# Autodesk Inventor assembly: Board
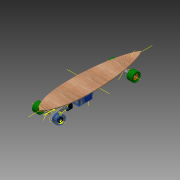
[picture p0: Inventor's stored thumbnail of the model, 180x180]
Saved by Autodesk Inventor 2015 (Build 190159000, 159)
## iProperties
Created: 2014-05-13
Part Number: Board
Document SubType Name: Assembly
Designer: dliu
Author: dliu
## Documents named in this file (9)
- C:\Users\dliu\Dropbox\dbhome\electric-longboard\dliu\DLiu Board.iam
- C:\Users\dliu\Dropbox\dbhome\electric-longboard\dliu\Board\Deck Pintail 9x37.iam
- C:\Users\dliu\Dropbox\dbhome\electric-longboard\dliu\Mount\Truck Caliber50 9in.iam
- C:\Users\dliu\Dropbox\dbhome\electric-longboard\dliu\Board\Wheel Blank Pro 83mm.ipt
- C:\Users\dliu\Dropbox\dbhome\electric-longboard\dliu\Mount\Mount.iam
- C:\Users\dliu\Dropbox\dbhome\electric-longboard\dliu\Electronics\Motor SK3 5065 275KV.ipt
- C:\Users\dliu\Dropbox\dbhome\electric-longboard\dliu\Pulleys\a_6a25m012df1506.ipt
- C:\Users\dliu\Dropbox\dbhome\electric-longboard\dliu\Wheel Insert\Wheel Insert Test Fit.iam
- C:\Users\dliu\Dropbox\dbhome\electric-longboard\dliu\Electronics\ElectronicsBox with components.iam
## Components (12 placed, 8 different names)
1. Deck Pintail 9x37:1 [sub-assembly] — Mate:1, Flush:3, Insert:3, Insert:4, Mate:19, Mate:20, Mate:21, Mate:26, Mate:28, Mate:29, Mate:30, Mate:31
2. Truck Caliber50 9in:1 [sub-assembly] — Mate:2, Mate:3, Mate:8, Mate:9, Mate:26, Mate:28, Mate:29, Mate:30, Mate:31
3. Truck Caliber50 9in:2 [sub-assembly] — Insert:3, Insert:4, Mate:4, Mate:5, Mate:6, Mate:7, Mate:12, Mate:13, Mate:14, Mate:19, Mate:20, Mate:21, Mate:34, Mate:35
4. Wheel Blank Pro 83mm:1 — Mate:2, Mate:3
5. Wheel Blank Pro 83mm:2 — Mate:8, Mate:9
6. Wheel Blank Pro 83mm:3 — Mate:6, Mate:7
7. Wheel Blank Pro 83mm:4 — Mate:4, Mate:5
8. Mount:1 [sub-assembly] — Mate:12, Mate:13, Mate:14, Mate:17, Mate:18, Mate:24
9. Motor SK3 5065 275KV:1 — Mate:17, Mate:18, Mate:22
10. a_6a25m012df1506:1 — Mate:22, Mate:24
11. Wheel Insert Test Fit:1 [sub-assembly] — Mate:34, Mate:35
12. ElectronicsBox with components:1 [sub-assembly]
## Relationships (29: Mate 26, Insert 2, Flush 1)
- Mate:1: Deck Pintail 9x37:1
- Flush:3: Deck Pintail 9x37:1
- Insert:3 (6.35 mm): Deck Pintail 9x37:1 ↔ Truck Caliber50 9in:2
- Insert:4 (6.35 mm): Deck Pintail 9x37:1 ↔ Truck Caliber50 9in:2
- Mate:2: Truck Caliber50 9in:1 ↔ Wheel Blank Pro 83mm:1
- Mate:3: Truck Caliber50 9in:1 ↔ Wheel Blank Pro 83mm:1
- Mate:4: Truck Caliber50 9in:2 ↔ Wheel Blank Pro 83mm:4
- Mate:5: Truck Caliber50 9in:2 ↔ Wheel Blank Pro 83mm:4
- Mate:6: Truck Caliber50 9in:2 ↔ Wheel Blank Pro 83mm:3
- Mate:7: Truck Caliber50 9in:2 ↔ Wheel Blank Pro 83mm:3
- Mate:8: Truck Caliber50 9in:1 ↔ Wheel Blank Pro 83mm:2
- Mate:9: Truck Caliber50 9in:1 ↔ Wheel Blank Pro 83mm:2
- Mate:12: Truck Caliber50 9in:2 ↔ Mount:1
- Mate:13: Truck Caliber50 9in:2 ↔ Mount:1
- Mate:14: Truck Caliber50 9in:2 ↔ Mount:1
- Mate:17: Mount:1 ↔ Motor SK3 5065 275KV:1
- Mate:18: Mount:1 ↔ Motor SK3 5065 275KV:1
- Mate:19: Deck Pintail 9x37:1 ↔ Truck Caliber50 9in:2
- Mate:20: Deck Pintail 9x37:1 ↔ Truck Caliber50 9in:2
- Mate:21: Deck Pintail 9x37:1 ↔ Truck Caliber50 9in:2
- Mate:22: Motor SK3 5065 275KV:1 ↔ a_6a25m012df1506:1
- Mate:24: Mount:1 ↔ a_6a25m012df1506:1
- Mate:26: Deck Pintail 9x37:1 ↔ Truck Caliber50 9in:1
- Mate:28 (0.4572 mm): Deck Pintail 9x37:1 ↔ Truck Caliber50 9in:1
- Mate:29 (0.4572 mm): Deck Pintail 9x37:1 ↔ Truck Caliber50 9in:1
- Mate:30 (0.4572 mm): Deck Pintail 9x37:1 ↔ Truck Caliber50 9in:1
- Mate:31 (0.4572 mm): Deck Pintail 9x37:1 ↔ Truck Caliber50 9in:1
- Mate:34: Truck Caliber50 9in:2 ↔ Wheel Insert Test Fit:1
- Mate:35: Truck Caliber50 9in:2 ↔ Wheel Insert Test Fit:1
